# Autodesk Inventor assembly: LOZYSKOWANIEdosprawdzenia
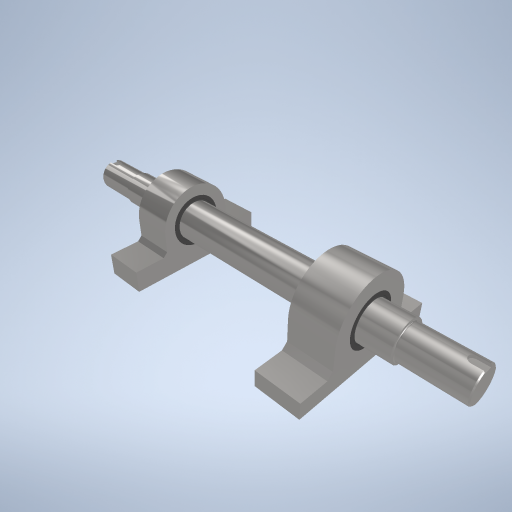
[picture p0: Inventor's stored thumbnail of the model, 512x512]
Saved by Autodesk Inventor 2024 (Build 280153000, 153)
## iProperties
Created: 2023-12-15
Part Number: LOZYSKOWANIEdosprawdzenia
Document SubType Name: Assembly
Designer: Wojciech
Author: Wojciech
## Documents named in this file (10)
- E:\studia\5sem\PKM\pkmp\MarcinPrabuckiPROJEKT3WAŁMASZYNOWY\LOZYSKOWANIEdosprawdzenia.iam
- E:\studia\5sem\PKM\pkmp\MarcinPrabuckiPROJEKT3WAŁMASZYNOWY\wał.ipt
- E:\studia\5sem\PKM\pkmp\MarcinPrabuckiPROJEKT3WAŁMASZYNOWY\LOZYSKOWANIE\Design Accelerator\Łożysko1.iam
- E:\studia\5sem\PKM\pkmp\MarcinPrabuckiPROJEKT3WAŁMASZYNOWY\LOZYSKOWANIE\Design Accelerator\Łożysko2.iam
- E:\studia\5sem\PKM\pkmp\MarcinPrabuckiPROJEKT3WAŁMASZYNOWY\LOZYSKOWANIE\ANSI B27.7 - 60(2).ipt
- E:\studia\5sem\PKM\pkmp\MarcinPrabuckiPROJEKT3WAŁMASZYNOWY\LOZYSKOWANIE\ANSI B27.7 - 70(2).ipt
- E:\studia\5sem\PKM\pkmp\MarcinPrabuckiPROJEKT3WAŁMASZYNOWY\obudowa Aa.ipt
- E:\studia\5sem\PKM\pkmp\MarcinPrabuckiPROJEKT3WAŁMASZYNOWY\ANSI B93.98M(3)\ANSI_B93.98M - 60x80x8-Typ 6.ipt
- E:\studia\5sem\PKM\pkmp\MarcinPrabuckiPROJEKT3WAŁMASZYNOWY\ANSI B93.98M(3)\ANSI_B93.98M - 70x90x10-Typ 6.ipt
- E:\studia\5sem\PKM\pkmp\MarcinPrabuckiPROJEKT3WAŁMASZYNOWY\obudowa B.ipt
## Components (12 placed, 8 different names)
1. wał:1 — Zestawiające:1, Zestawiające:2, Zestawiające:3, Zestawiające:4, Równoległe:1, Zestawiające:5, Zestawiające:6, Równoległe:4, Równoległe:5, Zestawiające:7, Zestawiające:8, Zestawiające:9, Zestawiające:10
2. Łożysko:1 [sub-assembly] — Zestawiające:1, Zestawiające:2, Równoległe:1, Równoległe:6, Równoległe:7, Kątowe:1
3. Łożysko:2 [sub-assembly] — Zestawiające:3, Zestawiające:4, Równoległe:2, Równoległe:3, Równoległe:8, Równoległe:11, Równoległe:12
4. Pierścień typu R 60:1 — Zestawiające:5, Zestawiające:6, Kątowe:1
5. Pierścień typu R 70:1 — Zestawiające:7, Zestawiające:9
6. Pierścień typu R 70:2 — Zestawiające:8, Zestawiające:10
7. obudowa Aa:1 — Równoległe:6, Równoległe:7, Wstawiające:1, Wstawiające:2
8. ANSI/B93.98M 60x80x8-Typ 6:1 — Wstawiające:2
9. ANSI/B93.98M 70x90x10-Typ 6:1 — Wstawiające:1
10. obudowa B:1 — Równoległe:9, Równoległe:10, Równoległe:11, Równoległe:13, Wstawiające:3, Równoległe:14
11. ANSI/B93.98M 70x90x10-Typ 6:2 — Wstawiające:3
12. ANSI/B93.98M 70x90x10-Typ 6:3 — Równoległe:14
## Relationships (28: Flush 14, Mate 10, Insert 3, Angle 1)
- Zestawiające:1 [Mate]: wał:1 ↔ Łożysko:1
- Zestawiające:2 [Mate]: wał:1 ↔ Łożysko:1
- Zestawiające:3 [Mate]: wał:1 ↔ Łożysko:2
- Zestawiające:4 [Mate]: wał:1 ↔ Łożysko:2
- Równoległe:1 [Flush]: wał:1 ↔ Łożysko:1
- Zestawiające:5 [Mate]: wał:1 ↔ Pierścień typu R 60:1
- Zestawiające:6 [Mate]: wał:1 ↔ Pierścień typu R 60:1
- Równoległe:2 [Flush]: Łożysko:2
- Równoległe:3 [Flush]: Łożysko:2
- Równoległe:4 [Flush]: wał:1
- Równoległe:5 [Flush]: wał:1
- Zestawiające:7 [Mate]: wał:1 ↔ Pierścień typu R 70:1
- Zestawiające:8 [Mate]: wał:1 ↔ Pierścień typu R 70:2
- Zestawiające:9 [Mate]: wał:1 ↔ Pierścień typu R 70:1
- Zestawiające:10 [Mate]: wał:1 ↔ Pierścień typu R 70:2
- Równoległe:6 [Flush]: Łożysko:1 ↔ obudowa Aa:1
- Równoległe:7 [Flush]: Łożysko:1 ↔ obudowa Aa:1
- Kątowe:1 [Angle] (0 deg): Łożysko:1 ↔ Pierścień typu R 60:1
- Wstawiające:1 [Insert]: obudowa Aa:1 ↔ ANSI/B93.98M 70x90x10-Typ 6:1
- Wstawiające:2 [Insert]: obudowa Aa:1 ↔ ANSI/B93.98M 60x80x8-Typ 6:1
- Równoległe:8 [Flush] (-12 mm): Łożysko:2
- Równoległe:9 [Flush]: obudowa B:1
- Równoległe:10 [Flush]: obudowa B:1
- Równoległe:11 [Flush]: Łożysko:2 ↔ obudowa B:1
- Równoległe:12 [Flush]: Łożysko:2
- Równoległe:13 [Flush]: obudowa B:1
- Wstawiające:3 [Insert]: obudowa B:1 ↔ ANSI/B93.98M 70x90x10-Typ 6:2
- Równoległe:14 [Flush]: obudowa B:1 ↔ ANSI/B93.98M 70x90x10-Typ 6:3
